# Autodesk Inventor assembly: PCBAssembly
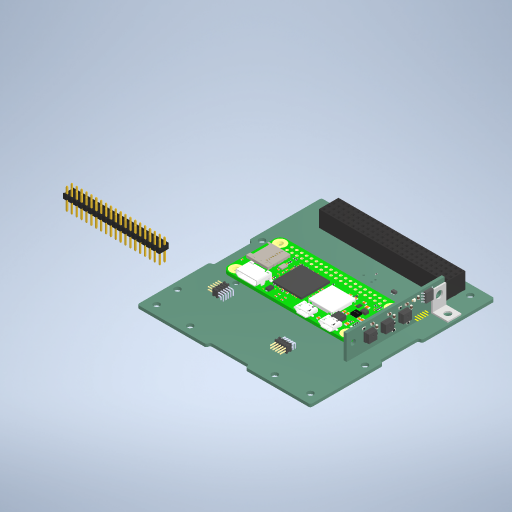
[picture p0: Inventor's stored thumbnail of the model, 512x512]
Saved by Autodesk Inventor 2023.5 (Build 275446020, 446B)
## iProperties
Created: 2026-07-20
Part Number: PCBAssembly
Document SubType Name: Assembly
Designer: User
Author: User
## Documents named in this file (5)
- C:\Users\User\Projects\missionpegasusPCB\CAD\PCBAssembly.iam
- C:\Users\User\Projects\missionpegasusPCB\CAD\615Bracket.ipt
- C:\Users\User\Projects\missionpegasusPCB\main-board\mainboard2\mainboard2.iam
- C:\Users\User\Projects\missionpegasusPCB\mezzanine-board\sensorboard3\sensorboard3.iam
- C:\Users\User\Downloads\User Library-40-pin GPIO Header for Raspberry Pi (color-coded)\User Library-40-pin GPIO Header for Raspberry Pi (color-coded).ipt
## Components (4 placed, 4 different names)
1. mainboard2:1 [sub-assembly] — Mate:1, Mate:2, Mate:4
2. 615Bracket:4 — Mate:3
3. sensorboard3:1 [sub-assembly] — Mate:1, Mate:2, Mate:3, Mate:4
4. User Library-40-pin GPIO Header for Raspberry Pi (color-coded):1
## Relationships (4: Mate 4)
- Mate:1: mainboard2:1 ↔ sensorboard3:1
- Mate:2: mainboard2:1 ↔ sensorboard3:1
- Mate:3: 615Bracket:4 ↔ sensorboard3:1
- Mate:4: mainboard2:1 ↔ sensorboard3:1
